# Autodesk Inventor assembly: Print 2
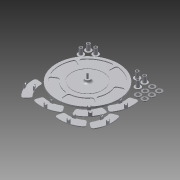
[picture p0: Inventor's stored thumbnail of the model, 180x180]
Saved by Autodesk Inventor 2014 (Build 180170000, 170)
## iProperties
Created: 2015-03-30
Part Number: Print 2
Document SubType Name: Assembly
Designer: MSI
Author: MSI
## Documents named in this file (5)
- C:\Users\MSI\Dropbox\Ingenieursproject\inventor\Print 2.iam
- C:\Users\MSI\Dropbox\Ingenieursproject\inventor\basis.ipt
- C:\Users\MSI\Dropbox\Ingenieursproject\inventor\Spoel kant.ipt
- C:\Users\MSI\Dropbox\Ingenieursproject\inventor\Spoel.ipt
- C:\Users\MSI\Dropbox\Ingenieursproject\inventor\spoelhouder.ipt
## Components (19 placed, 4 different names)
1. basis:1 — Mate:1
2. Spoel kant:1 — Mate:6
3. Spoel kant:2 — Mate:7
4. Spoel kant:3 — Mate:5
5. Spoel kant:4 — Mate:4
6. Spoel kant:5 — Mate:2
7. Spoel kant:6 — Mate:3
8. Spoel:1 — Mate:13
9. Spoel:2 — Mate:12
10. Spoel:3 — Mate:11
11. Spoel:4 — Mate:10
12. Spoel:5 — Mate:9
13. Spoel:6 — Mate:8
14. spoelhouder:1 — Mate:14
15. spoelhouder:2 — Mate:15
16. spoelhouder:3 — Mate:16
17. spoelhouder:4 — Mate:17
18. spoelhouder:5 — Mate:18
19. spoelhouder:6 — Mate:19
## Relationships (20: Mate 19, Flush 1)
- Flush:1
- Mate:1: basis:1
- Mate:2: Spoel kant:5
- Mate:3: Spoel kant:6
- Mate:4: Spoel kant:4
- Mate:5: Spoel kant:3
- Mate:6: Spoel kant:1
- Mate:7: Spoel kant:2
- Mate:8: Spoel:6
- Mate:9: Spoel:5
- Mate:10: Spoel:4
- Mate:11: Spoel:3
- Mate:12: Spoel:2
- Mate:13: Spoel:1
- Mate:14: spoelhouder:1
- Mate:15: spoelhouder:2
- Mate:16: spoelhouder:3
- Mate:17: spoelhouder:4
- Mate:18: spoelhouder:5
- Mate:19: spoelhouder:6
